# Autodesk Inventor assembly: 汎用脚ユニット
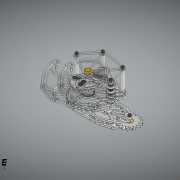
[picture p0: Inventor's stored thumbnail of the model, 180x180]
Saved by Autodesk Inventor 2020 (Build 240168000, 168)
## iProperties
Created: 2020-02-10
Part Number: 汎用脚ユニット
Document SubType Name: Assembly
Designer: tanjihayato
Author: tanjihayato
## Documents named in this file (26)
- \\Mac\Home\Documents\Inventor\2019お遊び機体\汎用脚ユニット.iam
- \\Mac\Home\Documents\Inventor\2019お遊び機体\後ろ脚内フレーム.ipt
- \\Mac\Home\Documents\Inventor\2019お遊び機体\後ろ脚内フレーム２.ipt
- \\Mac\Home\Documents\Inventor\2019お遊び機体\新型３ヘッケン_MIR.ipt
- \\Mac\Home\Documents\Inventor\2019お遊び機体\新型３揺動節_MIR.ipt
- \\Mac\Home\Documents\Inventor\2019お遊び機体\スペーサ　m3-l35.ipt
- \\Mac\Home\Documents\Inventor\2019お遊び機体\新型３脚最終段カム.ipt
- \\Mac\Home\Documents\Inventor\2019お遊び機体\後ろ脚外フレーム.ipt
- \\Mac\Home\Documents\Inventor\2019お遊び機体\z17ギア(インベンター).ipt
- \\Mac\Home\Documents\Inventor\2019お遊び機体\ベアリングフランジ6-12.ipt
- \\Mac\Home\Documents\Inventor\2019お遊び機体\z20ギア(インベンター).ipt
- \\Mac\Home\Documents\Inventor\2019お遊び機体\z28ギア(インベンター).ipt
- \\Mac\Home\Documents\Inventor\2019お遊び機体\スペーサ　m3-l6.ipt
- \\Mac\Home\Documents\Inventor\2019お遊び機体\脚ゴム.ipt
- \\Mac\Home\Documents\Inventor\2019お遊び機体\ベアリングH　d6-D10-B3.ipt
- \\Mac\Home\Documents\Inventor\2019お遊び機体\キャップボルトM3×8.ipt
- \\Mac\Home\Documents\Inventor\2019お遊び機体\フランジブッシュ　d12-14-F20.ipt
- \\Mac\Home\Documents\Inventor\2019お遊び機体\スペーサ　m3-l4.ipt
- \\Mac\Home\Documents\Inventor\2019お遊び機体\キャップボルトM3×20.ipt
- \\Mac\Home\Documents\Inventor\2019お遊び機体\後ろ脚内内フレーム.ipt
- \\Mac\Home\Documents\Inventor\2019お遊び機体\新型３クランク_MIR.ipt
- \\Mac\Home\Documents\Inventor\2019お遊び機体\新型３脚カム.ipt
- \\Mac\Home\Documents\Inventor\2019お遊び機体\新型３クランク根本_MIR.ipt
- \\Mac\Home\Documents\Inventor\2019お遊び機体\新型３涙_MIR.ipt
- \\Mac\Home\Documents\Inventor\2019お遊び機体\低頭ねじM4×8.ipt
- \\Mac\Home\Documents\Inventor\2019お遊び機体\フランジブッシュ　d6-D8-l5-h12.ipt
## Components (67 placed, 25 different names)
1. 後ろ脚内フレーム:1
2. 後ろ脚内フレーム２:1 — 挿入:47
3. 新型３ヘッケン_MIR:1
4. 新型３ヘッケン_MIR:2
5. 新型３ヘッケン_MIR:3
6. 新型３ヘッケン_MIR:4
7. 新型３揺動節_MIR:1 — 挿入:58
8. 新型３揺動節_MIR:2 — 挿入:60
9. 新型３揺動節_MIR:3 — 挿入:59
10. 新型３揺動節_MIR:4 — 挿入:61
11. スペーサ　m3-l35:1
12. スペーサ　m3-l35:2
13. スペーサ　m3-l35:3
14. スペーサ　m3-l35:4
15. 新型３脚最終段カム:1
16. 後ろ脚外フレーム:1
17. z17ギア(インベンター):1
18. ベアリングフランジ6-12:1
19. z20ギア(インベンター):1
20. z28ギア(インベンター):1 — 挿入:49, メイト:27
21. 新型３脚最終段カム:2
22. スペーサ　m3-l6:1
23. スペーサ　m3-l6:2
24. 脚ゴム:1
25. 脚ゴム:2
26. 脚ゴム:3
27. 脚ゴム:4
28. ベアリングH　d6-D10-B3:1
29. キャップボルトM3×8:1
30. キャップボルトM3×8:2
31. キャップボルトM3×8:3
32. キャップボルトM3×8:4
33. キャップボルトM3×8:5
34. キャップボルトM3×8:6
35. フランジブッシュ　d12-14-F20:1 — 挿入:47
36. スペーサ　m3-l4:1
37. キャップボルトM3×20:1
38. スペーサ　m3-l6:3
39. スペーサ　m3-l6:4
40. スペーサ　m3-l6:5
41. スペーサ　m3-l6:6
42. 後ろ脚内内フレーム:1 — 挿入:48, 挿入:62
43. キャップボルトM3×8:7
44. 新型３クランク_MIR:1 — 挿入:50, 挿入:51
45. 新型３クランク_MIR:2 — 挿入:54, 挿入:55
46. 新型３クランク_MIR:3 — 挿入:56, 挿入:57
47. 新型３脚カム:1
48. 新型３脚カム:2
49. 新型３脚カム:3
50. 新型３脚カム:4
51. 新型３クランク根本_MIR:1
52. 新型３涙_MIR:1 — 挿入:52, 挿入:53
53. フランジブッシュ　d12-14-F20:2 — 挿入:48
54. 新型３脚最終段カム:3 — 挿入:49, メイト:27
55. 低頭ねじM4×8:1 — 挿入:50
56. 低頭ねじM4×8:2 — 挿入:53
57. 低頭ねじM4×8:3 — 挿入:54
58. 低頭ねじM4×8:4 — 挿入:51
59. 低頭ねじM4×8:5 — 挿入:55
60. 低頭ねじM4×8:6 — 挿入:52
61. 低頭ねじM4×8:7 — 挿入:57
62. 低頭ねじM4×8:8 — 挿入:56
63. フランジブッシュ　d6-D8-l5-h12:1 — 挿入:58
64. フランジブッシュ　d6-D8-l5-h12:2 — 挿入:59
65. フランジブッシュ　d6-D8-l5-h12:3 — 挿入:61
66. フランジブッシュ　d6-D8-l5-h12:4 — 挿入:60
67. スペーサ　m3-l6:7 — 挿入:62
## Relationships (92: Insert 61, Mate 27, Flush 4)
- [Insert]: 後ろ脚内フレーム:1 ↔ 後ろ脚内フレーム２:1
- [Mate]: 後ろ脚内フレーム:1 ↔ 後ろ脚内フレーム２:1
- [Insert] (0.25 mm): 新型３ヘッケン_MIR:1 ↔ 新型３クランク根本_MIR:1
- [Insert] (0.25 mm): 新型３ヘッケン_MIR:2 ↔ 新型３クランク_MIR:3
- [Insert] (0.25 mm): 新型３ヘッケン_MIR:3 ↔ 新型３クランク_MIR:2
- [Insert] (0.25 mm): 新型３ヘッケン_MIR:4 ↔ 新型３クランク_MIR:1
- [Insert]: 新型３ヘッケン_MIR:4 ↔ 新型３揺動節_MIR:1
- [Insert]: 新型３ヘッケン_MIR:2 ↔ 新型３揺動節_MIR:2
- [Insert]: 新型３ヘッケン_MIR:3 ↔ 新型３揺動節_MIR:3
- [Insert]: 新型３ヘッケン_MIR:1 ↔ 新型３揺動節_MIR:4
- [Insert]: 後ろ脚内フレーム２:1 ↔ スペーサ　m3-l35:2
- [Insert]: 後ろ脚内フレーム２:1 ↔ スペーサ　m3-l35:1
- [Insert]: 後ろ脚内フレーム２:1 ↔ スペーサ　m3-l35:4
- [Insert]: 後ろ脚内フレーム２:1 ↔ スペーサ　m3-l35:3
- [Insert]: 新型３脚最終段カム:1 ↔ 新型３クランク根本_MIR:1
- [Mate]: 新型３脚最終段カム:1 ↔ 新型３クランク根本_MIR:1
- [Mate]: 新型３揺動節_MIR:4 ↔ スペーサ　m3-l35:3
- [Mate]: 新型３揺動節_MIR:1 ↔ スペーサ　m3-l35:3
- [Mate]: 新型３揺動節_MIR:3 ↔ スペーサ　m3-l35:3
- [Mate]: 新型３揺動節_MIR:2 ↔ スペーサ　m3-l35:3
- [Insert]: スペーサ　m3-l35:3 ↔ 後ろ脚外フレーム:1
- [Mate]: スペーサ　m3-l35:1 ↔ 後ろ脚外フレーム:1
- [Insert]: z17ギア(インベンター):1 ↔ ベアリングフランジ6-12:1
- [Insert] (1 mm): 後ろ脚内フレーム:1 ↔ ベアリングフランジ6-12:1
- [Insert]: 新型３脚最終段カム:1 ↔ 新型３脚最終段カム:2
- [Mate]: 新型３脚最終段カム:1 ↔ 新型３脚最終段カム:2
- [Insert]: z28ギア(インベンター):1 ↔ 新型３脚最終段カム:2
- [Mate]: z28ギア(インベンター):1 ↔ 新型３脚最終段カム:2
- [Insert]: 後ろ脚内フレーム:1 ↔ スペーサ　m3-l6:1
- [Insert]: 後ろ脚内フレーム:1 ↔ スペーサ　m3-l6:2
- [Mate]: 新型３ヘッケン_MIR:2 ↔ 脚ゴム:4
- [Mate]: 新型３ヘッケン_MIR:2 ↔ 脚ゴム:4
- [Flush]: 新型３ヘッケン_MIR:2 ↔ 脚ゴム:4
- [Mate]: 新型３ヘッケン_MIR:1 ↔ 脚ゴム:3
- [Mate]: 新型３ヘッケン_MIR:1 ↔ 脚ゴム:3
- [Flush]: 新型３ヘッケン_MIR:1 ↔ 脚ゴム:3
- [Mate]: 新型３ヘッケン_MIR:3 ↔ 脚ゴム:1
- [Mate]: 新型３ヘッケン_MIR:3 ↔ 脚ゴム:1
- [Flush]: 新型３ヘッケン_MIR:3 ↔ 脚ゴム:1
- [Mate]: 新型３ヘッケン_MIR:4 ↔ 脚ゴム:2
- [Mate]: 新型３ヘッケン_MIR:4 ↔ 脚ゴム:2
- [Flush]: 新型３ヘッケン_MIR:4 ↔ 脚ゴム:2
- [Insert]: 後ろ脚内フレーム２:1 ↔ キャップボルトM3×8:1
- [Insert]: 後ろ脚内フレーム２:1 ↔ キャップボルトM3×8:2
- [Insert]: 後ろ脚外フレーム:1 ↔ キャップボルトM3×8:3
- [Insert]: 後ろ脚外フレーム:1 ↔ キャップボルトM3×8:6
- [Insert]: 後ろ脚外フレーム:1 ↔ キャップボルトM3×8:5
- [Insert]: 後ろ脚外フレーム:1 ↔ キャップボルトM3×8:4
- [Insert]: 後ろ脚内フレーム:1 ↔ スペーサ　m3-l4:1
- [Insert]: 後ろ脚内フレーム:1 ↔ スペーサ　m3-l6:6
- [Insert]: 後ろ脚内フレーム:1 ↔ スペーサ　m3-l6:5
- [Insert]: 後ろ脚内フレーム:1 ↔ スペーサ　m3-l6:4
- [Insert]: 後ろ脚内フレーム:1 ↔ スペーサ　m3-l6:3
- [Insert]: スペーサ　m3-l4:1 ↔ キャップボルトM3×20:1
- [Insert]: スペーサ　m3-l6:5 ↔ 後ろ脚内内フレーム:1
- [Mate]: スペーサ　m3-l6:6 ↔ 後ろ脚内内フレーム:1
- [Insert]: 後ろ脚内フレーム２:1 ↔ キャップボルトM3×8:7
- [Insert]: 後ろ脚外フレーム:1 ↔ ベアリングH　d6-D10-B3:1
- [Insert] (-0.5 mm): 後ろ脚内フレーム２:1 ↔ 新型３脚最終段カム:1
- [Mate]: 新型３クランク_MIR:1 ↔ 新型３脚カム:1
- [Insert]: 新型３クランク_MIR:1 ↔ 新型３脚カム:1
- [Mate]: 新型３クランク_MIR:1 ↔ 新型３脚カム:2
- [Insert]: 新型３クランク_MIR:1 ↔ 新型３脚カム:2
- [Mate]: 新型３クランク_MIR:2 ↔ 新型３脚カム:2
- [Insert]: 新型３クランク_MIR:2 ↔ 新型３脚カム:2
- [Mate]: 新型３クランク_MIR:2 ↔ 新型３脚カム:3
- [Insert]: 新型３クランク_MIR:2 ↔ 新型３脚カム:3
- [Mate]: 新型３クランク_MIR:3 ↔ 新型３脚カム:3
- [Insert]: 新型３クランク_MIR:3 ↔ 新型３脚カム:3
- [Mate]: 新型３クランク_MIR:3 ↔ 新型３脚カム:4
- [Insert]: 新型３クランク_MIR:3 ↔ 新型３脚カム:4
- [Mate]: 新型３脚カム:4 ↔ 新型３クランク根本_MIR:1
- [Insert]: 新型３脚カム:4 ↔ 新型３クランク根本_MIR:1
- [Mate]: 新型３脚カム:1 ↔ 新型３涙_MIR:1
- [Insert]: 新型３脚カム:1 ↔ 新型３涙_MIR:1
- 挿入:47 [Insert]: 後ろ脚内フレーム２:1 ↔ フランジブッシュ　d12-14-F20:1
- 挿入:48 [Insert]: 後ろ脚内内フレーム:1 ↔ フランジブッシュ　d12-14-F20:2
- 挿入:49 [Insert]: z28ギア(インベンター):1 ↔ 新型３脚最終段カム:3
- メイト:27 [Mate]: z28ギア(インベンター):1 ↔ 新型３脚最終段カム:3
- 挿入:50 [Insert]: 新型３クランク_MIR:1 ↔ 低頭ねじM4×8:1
- 挿入:51 [Insert]: 新型３クランク_MIR:1 ↔ 低頭ねじM4×8:4
- 挿入:52 [Insert]: 新型３涙_MIR:1 ↔ 低頭ねじM4×8:6
- 挿入:53 [Insert]: 新型３涙_MIR:1 ↔ 低頭ねじM4×8:2
- 挿入:54 [Insert]: 新型３クランク_MIR:2 ↔ 低頭ねじM4×8:3
- 挿入:55 [Insert]: 新型３クランク_MIR:2 ↔ 低頭ねじM4×8:5
- 挿入:56 [Insert]: 新型３クランク_MIR:3 ↔ 低頭ねじM4×8:8
- 挿入:57 [Insert]: 新型３クランク_MIR:3 ↔ 低頭ねじM4×8:7
- 挿入:58 [Insert]: 新型３揺動節_MIR:1 ↔ フランジブッシュ　d6-D8-l5-h12:1
- 挿入:59 [Insert]: 新型３揺動節_MIR:3 ↔ フランジブッシュ　d6-D8-l5-h12:2
- 挿入:60 [Insert]: 新型３揺動節_MIR:2 ↔ フランジブッシュ　d6-D8-l5-h12:4
- 挿入:61 [Insert]: 新型３揺動節_MIR:4 ↔ フランジブッシュ　d6-D8-l5-h12:3
- 挿入:62 [Insert]: 後ろ脚内内フレーム:1 ↔ スペーサ　m3-l6:7
## Named parameters: d189_d187 = 0 mm, d48_d72 = 0 mm, d49_d73 = 0 mm, d50_d75 = 0.25 mm
